# Autodesk Inventor assembly: elevation_assembly_blacha_gieta
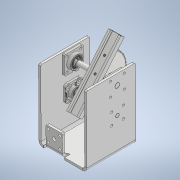
[picture p0: Inventor's stored thumbnail of the model, 180x180]
Saved by Autodesk Inventor 2020 (Build 240168000, 168)
## iProperties
Created: 2020-08-26
Part Number: elevation_assembly_blacha_gieta
Document SubType Name: Assembly
Designer: Hesekiel
Author: Hesekiel
## Documents named in this file (13)
- C:\Users\Hesekiel\Desktop\Equatorial-Mount-MUM\Mechanika\Mechanizm elewacji Filip\CAD\elevation_assembly_blacha_gieta.iam
- C:\Users\Hesekiel\Desktop\Equatorial-Mount-MUM\Mechanika\Mechanizm elewacji Filip\CAD\baza_blacha_gięta.ipt
- C:\Users\Hesekiel\Desktop\Equatorial-Mount-MUM\Mechanika\Mechanizm elewacji Filip\CAD\F4BSS 20M-YTPSS\F4BSS 20M-YTPSS.iam
- C:\Users\Hesekiel\Desktop\Equatorial-Mount-MUM\Mechanika\Mechanizm elewacji Filip\CAD\wał_uzębienia.ipt
- C:\Users\Hesekiel\Desktop\Equatorial-Mount-MUM\Mechanika\Mechanizm elewacji Filip\CAD\rack_and_pinion.iam
- C:\Users\Hesekiel\Desktop\Equatorial-Mount-MUM\Mechanika\Mechanizm elewacji Filip\CAD\wał_półkola.ipt
- C:\Users\Hesekiel\Desktop\Equatorial-Mount-MUM\Mechanika\Mechanizm elewacji Filip\CAD\M6x6_DIN914.ipt
- C:\Users\Hesekiel\Desktop\Equatorial-Mount-MUM\Mechanika\Uchwyty, elementy i inne\szyna.ipt
- C:\Users\Hesekiel\Desktop\Equatorial-Mount-MUM\Mechanika\Mechanizm elewacji Filip\CAD\FY 15 FM\FY 15 FM.iam
- C:\Users\Hesekiel\Desktop\Equatorial-Mount-MUM\Mechanika\Mechanizm elewacji Filip\CAD\uchwyt_szyny.ipt
- C:\Users\Hesekiel\Desktop\Equatorial-Mount-MUM\Mechanika\Mechanizm elewacji Filip\CAD\elevation_assembly_blacha_gieta\Design Accelerator\Bolted Connection1.iam
- C:\Users\Hesekiel\Desktop\Equatorial-Mount-MUM\Mechanika\Mechanizm elewacji Filip\CAD\elevation_assembly_blacha_gieta\Design Accelerator\Bolted Connection2.iam
- C:\Users\Hesekiel\Desktop\Equatorial-Mount-MUM\Mechanika\Mechanizm elewacji Filip\CAD\elevation_assembly_blacha_gieta\Design Accelerator\Bolted Connection3.iam
## Components (14 placed, 10 different names)
1. baza_blacha_gięta:1 — Mate:1, Mate:2, Mate:3, Mate:4, Mate:5, Mate:6, Flush:1, Mate:23, Flush:2, Rotational:1, Rotational:2, Mate:25, Mate:26, Mate:27, Mate:28, Mate:29, Mate:30
2. F4BSS 20M-YTPSS:1 [sub-assembly] — Mate:4, Mate:5, Mate:6
3. F4BSS 20M-YTPSS:2 [sub-assembly] — Mate:1, Mate:2, Mate:3
4. wał_uzębienia:1 — Flush:1, Mate:21, Mate:22, Rotational:2, Rigid:1
5. rack_and_pinion:1 [sub-assembly] — Mate:21, Mate:22, Mate:24, Rigid:2
6. wał_półkola:1 — Mate:23, Flush:2, Rotational:1, Mate:24
7. M6x6_DIN914:1 — Rigid:1
8. szyna:1 — Rigid:3
9. FY 15 FM:1 [sub-assembly] — Mate:25, Mate:26, Mate:27
10. FY 15 FM:2 [sub-assembly] — Mate:28, Mate:29, Mate:30
11. uchwyt_szyny:1 — Rigid:2, Rigid:3, Mate:31, Mate:32, Mate:33, Mate:34, Mate:35, Mate:36
12. Bolted Connection:1 [sub-assembly] — Mate:31, Mate:32
13. Bolted Connection:2 [sub-assembly] — Mate:33, Mate:34
14. Bolted Connection:3 [sub-assembly] — Mate:35, Mate:36
## Relationships (29: Mate 22, WeldJoint 3, Flush 2, RevoluteJoint 2)
- Mate:1: baza_blacha_gięta:1 ↔ F4BSS 20M-YTPSS:2
- Mate:2: baza_blacha_gięta:1 ↔ F4BSS 20M-YTPSS:2
- Mate:3: baza_blacha_gięta:1 ↔ F4BSS 20M-YTPSS:2
- Mate:4: baza_blacha_gięta:1 ↔ F4BSS 20M-YTPSS:1
- Mate:5: baza_blacha_gięta:1 ↔ F4BSS 20M-YTPSS:1
- Mate:6: baza_blacha_gięta:1 ↔ F4BSS 20M-YTPSS:1
- Flush:1: baza_blacha_gięta:1 ↔ wał_uzębienia:1
- Mate:21: wał_uzębienia:1 ↔ rack_and_pinion:1
- Mate:22: wał_uzębienia:1 ↔ rack_and_pinion:1
- Mate:23: baza_blacha_gięta:1 ↔ wał_półkola:1
- Flush:2: baza_blacha_gięta:1 ↔ wał_półkola:1
- Rotational:1 [RevoluteJoint]: baza_blacha_gięta:1 ↔ wał_półkola:1
- Rotational:2 [RevoluteJoint]: baza_blacha_gięta:1 ↔ wał_uzębienia:1
- Mate:24: rack_and_pinion:1 ↔ wał_półkola:1
- Rigid:1 [WeldJoint]: wał_uzębienia:1 ↔ M6x6_DIN914:1
- Mate:25: baza_blacha_gięta:1 ↔ FY 15 FM:1
- Mate:26: baza_blacha_gięta:1 ↔ FY 15 FM:1
- Mate:27: baza_blacha_gięta:1 ↔ FY 15 FM:1
- Mate:28: baza_blacha_gięta:1 ↔ FY 15 FM:2
- Mate:29: baza_blacha_gięta:1 ↔ FY 15 FM:2
- Mate:30: baza_blacha_gięta:1 ↔ FY 15 FM:2
- Rigid:2 [WeldJoint]: rack_and_pinion:1 ↔ uchwyt_szyny:1
- Rigid:3 [WeldJoint]: szyna:1 ↔ uchwyt_szyny:1
- Mate:31: uchwyt_szyny:1 ↔ Bolted Connection:1
- Mate:32: uchwyt_szyny:1 ↔ Bolted Connection:1
- Mate:33: uchwyt_szyny:1 ↔ Bolted Connection:2
- Mate:34: uchwyt_szyny:1 ↔ Bolted Connection:2
- Mate:35: uchwyt_szyny:1 ↔ Bolted Connection:3
- Mate:36: uchwyt_szyny:1 ↔ Bolted Connection:3
